# Autodesk Inventor assembly: konsol
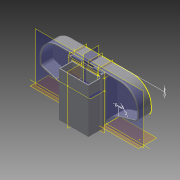
[picture p0: Inventor's stored thumbnail of the model, 180x180]
Saved by Autodesk Inventor 2015 (Build 190159000, 159)
## iProperties
Created: 2015-12-13
Part Number: konsol
Document SubType Name: Assembly
Designer: abberik
Author: abberik
## Documents named in this file (4)
- E:\bibliotek\dokument\Raspberry Pi gaming konsol\konsol.iam
- E:\bibliotek\dokument\Raspberry Pi gaming konsol\kontroller3.ipt
- E:\bibliotek\dokument\Raspberry Pi gaming konsol\PI_Skal_med_rals.ipt
- E:\bibliotek\dokument\Raspberry Pi gaming konsol\batteri.ipt
## Components (3 placed, 3 different names)
1. kontroller3:1 — Mate:1, Mate:2, Flush:1, Mate:3, Mate:4
2. PI_Skal_med_rals:1 — Mate:1, Mate:2, Flush:1
3. batteri:1 — Mate:3, Mate:4
## Relationships (5: Mate 4, Flush 1)
- Mate:1: kontroller3:1 ↔ PI_Skal_med_rals:1
- Mate:2: kontroller3:1 ↔ PI_Skal_med_rals:1
- Flush:1: kontroller3:1 ↔ PI_Skal_med_rals:1
- Mate:3: kontroller3:1 ↔ batteri:1
- Mate:4: kontroller3:1 ↔ batteri:1
